# Autodesk Inventor assembly: Base2
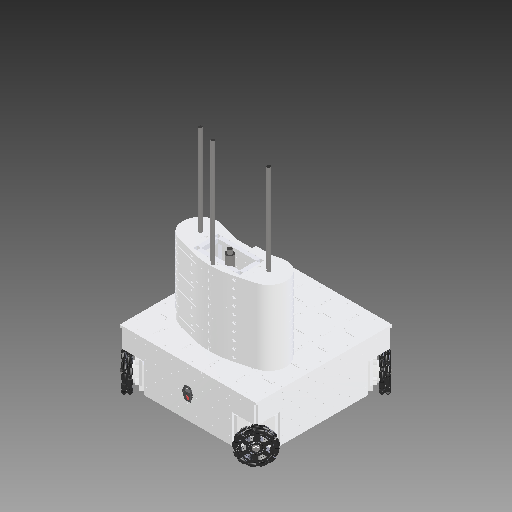
[picture p0: Inventor's stored thumbnail of the model, 512x512]
Saved by Autodesk Inventor 2017 SP1 (Build 210196100, 196)
## iProperties
Created: 2017-06-13
Part Number: Base2
Document SubType Name: Assembly
Designer: zallen
Author: zallen
## Documents named in this file (13)
- C:\Users\Zach\Documents\GitHub\cr-laundry-robot\src\Base\Base.iam
- C:\Users\Zach\Documents\GitHub\cr-laundry-robot\src\Base\Chassis\Chassis.iam
- C:\Users\Zach\Documents\GitHub\cr-laundry-robot\lib\Linear Actuator 450mm\LinearActuator450mm.iam
- C:\Users\Zach\Documents\GitHub\cr-laundry-robot\src\Base\Wheel Assembly\Wheel Assembly.iam
- C:\Users\Zach\Documents\GitHub\cr-laundry-robot\src\Base\Quick Shaft 12mm x 500mm.ipt
- C:\Users\Zach\Documents\GitHub\cr-laundry-robot\src\Base\Rod End Stop.ipt
- C:\Users\Zach\Documents\GitHub\cr-laundry-robot\lib\ExpertPower EXP12180 Battery.ipt
- C:\Users\Zach\Documents\GitHub\cr-laundry-robot\src\Base\Battery Box\BatteryBox.iam
- C:\Users\Zach\Documents\GitHub\cr-laundry-robot\src\Base\Side Panel\Side Panel.iam
- C:\Users\Zach\Documents\GitHub\cr-laundry-robot\src\Base\Side Panel\Side Panel Front.iam
- C:\Users\Zach\Documents\GitHub\cr-laundry-robot\src\Base\Side Panel\Side Panel Back.iam
- C:\Users\Zach\Documents\GitHub\cr-laundry-robot\src\Base\Rise Base Assembly\Riser Base.iam
- C:\Users\Zach\Documents\GitHub\cr-laundry-robot\src\Base\Top Cover Assembly\Top Cover Assembly.iam
## Components (18 placed, 12 different names)
1. Chassis:1 [sub-assembly] — Mate:17, Mate:36, Mate:37, Mate:38, Mate:39, Mate:40, Mate:41, Mate:42, Mate:43, Mate:44, Mate:45, Mate:46, Mate:47, Mate:48, Mate:49, Mate:165, Flush:63, Mate:166, Flush:64, Mate:168, Mate:169, Mate:174, Mate:175, Mate:176, Mate:177, Mate:178, Mate:179, Mate:181, Mate:184, Mate:185
2. LinearActuator450mm:1 [sub-assembly] — Mate:17
3. Wheel Assembly:1 [sub-assembly] — Mate:36, Mate:37, Mate:38, Mate:39, Mate:40
4. Wheel Assembly:2 [sub-assembly] — Mate:41, Mate:42, Mate:43
5. Wheel Assembly:3 [sub-assembly] — Mate:44, Mate:45, Mate:46
6. Wheel Assembly:4 [sub-assembly] — Mate:47, Mate:48, Mate:49
7. Quick Shaft 12mm x 500mm:1 — Flush:62, Mate:172, Mate:187, Mate:195
8. Quick Shaft 12mm x 500mm:2 — Flush:62, Mate:173, Mate:186, Mate:196
9. Quick Shaft 12mm x 500mm:3 — Mate:163, Mate:170, Mate:188, Mate:189
10. Rod End Stop:1 — Mate:163, Mate:189, Mate:192
11. ExpertPower EXP12180 Battery:1 — Mate:165, Mate:167, Mate:168
12. BatteryBox:1 [sub-assembly] — Flush:63, Mate:166, Flush:64, Mate:167
13. Side Panel:3 [sub-assembly] — Mate:174, Mate:175, Mate:193
14. Side Panel:4 [sub-assembly] — Mate:178, Mate:179, Mate:180
15. Side Panel Front:1 [sub-assembly] — Mate:176, Mate:177
16. Side Panel Back:1 [sub-assembly] — Mate:180, Mate:181, Mate:194
17. Riser Base:1 [sub-assembly] — Mate:184, Mate:185, Mate:186, Mate:187, Mate:188
18. Top Cover Assembly:1 [sub-assembly] — Mate:192, Mate:193, Mate:194, Mate:195, Mate:196
## Relationships (46: Mate 43, Flush 3)
- Mate:17: Chassis:1 ↔ LinearActuator450mm:1
- Mate:36: Chassis:1 ↔ Wheel Assembly:1
- Mate:37: Chassis:1 ↔ Wheel Assembly:1
- Mate:38: Chassis:1 ↔ Wheel Assembly:1
- Mate:39: Chassis:1 ↔ Wheel Assembly:1
- Mate:40: Chassis:1 ↔ Wheel Assembly:1
- Mate:41: Chassis:1 ↔ Wheel Assembly:2
- Mate:42: Chassis:1 ↔ Wheel Assembly:2
- Mate:43: Chassis:1 ↔ Wheel Assembly:2
- Mate:44: Chassis:1 ↔ Wheel Assembly:3
- Mate:45: Chassis:1 ↔ Wheel Assembly:3
- Mate:46: Chassis:1 ↔ Wheel Assembly:3
- Mate:47: Chassis:1 ↔ Wheel Assembly:4
- Mate:48: Chassis:1 ↔ Wheel Assembly:4
- Mate:49: Chassis:1 ↔ Wheel Assembly:4
- Flush:62: Quick Shaft 12mm x 500mm:1 ↔ Quick Shaft 12mm x 500mm:2
- Mate:163: Quick Shaft 12mm x 500mm:3 ↔ Rod End Stop:1
- Mate:165: Chassis:1 ↔ ExpertPower EXP12180 Battery:1
- Flush:63: Chassis:1 ↔ BatteryBox:1
- Mate:166: Chassis:1 ↔ BatteryBox:1
- Flush:64: Chassis:1 ↔ BatteryBox:1
- Mate:167: ExpertPower EXP12180 Battery:1 ↔ BatteryBox:1
- Mate:168: Chassis:1 ↔ ExpertPower EXP12180 Battery:1
- Mate:169: Chassis:1
- Mate:170: Quick Shaft 12mm x 500mm:3
- Mate:172: Quick Shaft 12mm x 500mm:1
- Mate:173: Quick Shaft 12mm x 500mm:2
- Mate:174: Chassis:1 ↔ Side Panel:3
- Mate:175: Chassis:1 ↔ Side Panel:3
- Mate:176: Chassis:1 ↔ Side Panel Front:1
- Mate:177: Chassis:1 ↔ Side Panel Front:1
- Mate:178: Chassis:1 ↔ Side Panel:4
- Mate:179: Chassis:1 ↔ Side Panel:4
- Mate:180: Side Panel:4 ↔ Side Panel Back:1
- Mate:181: Chassis:1 ↔ Side Panel Back:1
- Mate:184: Chassis:1 ↔ Riser Base:1
- Mate:185: Chassis:1 ↔ Riser Base:1
- Mate:186: Quick Shaft 12mm x 500mm:2 ↔ Riser Base:1
- Mate:187: Quick Shaft 12mm x 500mm:1 ↔ Riser Base:1
- Mate:188: Quick Shaft 12mm x 500mm:3 ↔ Riser Base:1
- Mate:189: Quick Shaft 12mm x 500mm:3 ↔ Rod End Stop:1
- Mate:192: Rod End Stop:1 ↔ Top Cover Assembly:1
- Mate:193: Side Panel:3 ↔ Top Cover Assembly:1
- Mate:194: Side Panel Back:1 ↔ Top Cover Assembly:1
- Mate:195: Quick Shaft 12mm x 500mm:1 ↔ Top Cover Assembly:1
- Mate:196: Quick Shaft 12mm x 500mm:2 ↔ Top Cover Assembly:1
